# Autodesk Inventor assembly: Frame
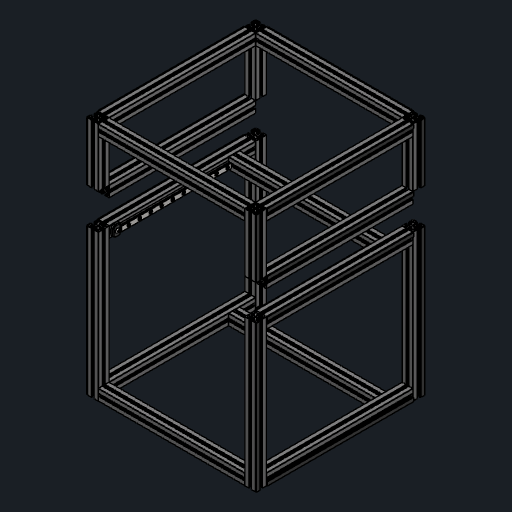
[picture p0: Inventor's stored thumbnail of the model, 512x512]
Saved by Autodesk Inventor 2026 (Build 300175050, 175E)
## iProperties
Created: 2025-05-09
Part Number: Frame
Document SubType Name: Assembly
Designer: AdminForWorker
Title: Frame
Author: AdminForWorker
## Documents named in this file (7)
- C:\Users\Joshua Eah\Documents\GitHub\Voron-0\CAD\Master Assembly\Frame\Frame.iam
- C:\Users\Joshua Eah\Documents\GitHub\Voron-0\CAD\Master Assembly\Linear Rail\MGN7 Rail 150mm.iam
- MGN7 150mm Rail.iam
- C:\Users\Joshua Eah\Documents\GitHub\Voron-0\CAD\Master Assembly\Frame\Subassemblies\Rail Stop.iam
- C:\Users\Joshua Eah\Documents\GitHub\Voron-0\CAD\Master Assembly\Frame\Subassemblies\Frame Extrusions.iam
- Extrusions.iam
- C:\Users\Joshua Eah\Documents\GitHub\Voron-0\CAD\Master Assembly\Frame\Foam Tape.iam
## Components (6 placed, 4 different names)
1. Extrusions:1 [sub-assembly]
2. MGN7 150mm Rail:3 [sub-assembly] — Mate:20
3. MGN7 150mm Rail:4 [sub-assembly] — Mate:22
4. Rail Stop:1 [sub-assembly] — Mate:20
5. Rail Stop:2 [sub-assembly] — Mate:22
6. Foam Tape:1 [sub-assembly]
## Relationships (99: Flush 62, Mate 37)
- [Mate]: Extrusions:1 ↔ MGN7 150mm Rail:3
- [Mate] (0.1 mm): Extrusions:1 ↔ MGN7 150mm Rail:3
- [Flush] (38 mm): Extrusions:1 ↔ MGN7 150mm Rail:3
- [Flush] (38 mm): Extrusions:1 ↔ MGN7 150mm Rail:4
- [Mate]: Extrusions:1 ↔ MGN7 150mm Rail:4
- [Mate] (0.1 mm): Extrusions:1 ↔ MGN7 150mm Rail:4
- [Mate]: Extrusions:1 ↔ Rail Stop:1
- Mate:20: MGN7 150mm Rail:3 ↔ Rail Stop:1
- [Flush]: Extrusions:1 ↔ Rail Stop:1
- [Mate]: Extrusions:1 ↔ Rail Stop:2
- Mate:22: MGN7 150mm Rail:4 ↔ Rail Stop:2
- [Flush]: Extrusions:1 ↔ Rail Stop:2
- [Mate]: Extrusions:1 ↔ Foam Tape:1
- [Flush]: Extrusions:1 ↔ Foam Tape:1
- [Mate]: Extrusions:1 ↔ Foam Tape:1
- [Flush]: Extrusions:1 ↔ Foam Tape:1
- [Mate]: Extrusions:1 ↔ Foam Tape:1
- [Flush]: Extrusions:1 ↔ Foam Tape:1
- [Mate]: Extrusions:1 ↔ Foam Tape:1
- [Flush]: Extrusions:1 ↔ Foam Tape:1
- [Mate]: Extrusions:1 ↔ Foam Tape:1
- [Flush]: Extrusions:1 ↔ Foam Tape:1
- [Flush]: Extrusions:1 ↔ Foam Tape:1
- [Mate]: Extrusions:1 ↔ Foam Tape:1
- [Flush]: Extrusions:1 ↔ Foam Tape:1
- [Flush]: Extrusions:1 ↔ Foam Tape:1
- [Mate]: Extrusions:1 ↔ Foam Tape:1
- [Flush]: Extrusions:1 ↔ Foam Tape:1
- [Flush]: Extrusions:1 ↔ Foam Tape:1
- [Mate]: Extrusions:1 ↔ Foam Tape:1
- [Flush]: Extrusions:1 ↔ Foam Tape:1
- [Flush]: Extrusions:1 ↔ Foam Tape:1
- [Mate]: Extrusions:1 ↔ Foam Tape:1
- [Flush]: Extrusions:1 ↔ Foam Tape:1
- [Flush]: Extrusions:1 ↔ Foam Tape:1
- [Mate]: Extrusions:1 ↔ Foam Tape:1
- [Flush]: Extrusions:1 ↔ Foam Tape:1
- [Flush]: Extrusions:1 ↔ Foam Tape:1
- [Mate]: Extrusions:1 ↔ Foam Tape:1
- [Flush]: Extrusions:1 ↔ Foam Tape:1
- [Flush]: Extrusions:1 ↔ Foam Tape:1
- [Mate]: Extrusions:1 ↔ Foam Tape:1
- [Flush]: Extrusions:1 ↔ Foam Tape:1
- [Flush]: Extrusions:1 ↔ Foam Tape:1
- [Flush]: Extrusions:1 ↔ Foam Tape:1
- [Flush]: Extrusions:1 ↔ Foam Tape:1
- [Mate]: Extrusions:1 ↔ Foam Tape:1
- [Flush]: Extrusions:1 ↔ Foam Tape:1
- [Flush]: Extrusions:1 ↔ Foam Tape:1
- [Mate]: Extrusions:1 ↔ Foam Tape:1
- [Flush]: Extrusions:1 ↔ Foam Tape:1
- [Flush]: Extrusions:1 ↔ Foam Tape:1
- [Flush]: Extrusions:1 ↔ Foam Tape:1
- [Flush]: Extrusions:1 ↔ Foam Tape:1
- [Mate]: Extrusions:1 ↔ Foam Tape:1
- [Flush]: Extrusions:1 ↔ Foam Tape:1
- [Flush]: Extrusions:1 ↔ Foam Tape:1
- [Mate]: Extrusions:1 ↔ Foam Tape:1
- [Flush]: Extrusions:1 ↔ Foam Tape:1
- [Flush]: Extrusions:1 ↔ Foam Tape:1
- [Mate]: Extrusions:1 ↔ Foam Tape:1
- [Flush]: Extrusions:1 ↔ Foam Tape:1
- [Flush]: Extrusions:1 ↔ Foam Tape:1
- [Mate]: Extrusions:1 ↔ Foam Tape:1
- [Flush]: Extrusions:1 ↔ Foam Tape:1
- [Flush]: Extrusions:1 ↔ Foam Tape:1
- [Mate]: Extrusions:1 ↔ Foam Tape:1
- [Flush]: Extrusions:1 ↔ Foam Tape:1
- [Flush]: Extrusions:1 ↔ Foam Tape:1
- [Mate]: Extrusions:1 ↔ Foam Tape:1
- [Flush]: Extrusions:1 ↔ Foam Tape:1
- [Flush]: Extrusions:1 ↔ Foam Tape:1
- [Mate]: Extrusions:1 ↔ Foam Tape:1
- [Flush]: Extrusions:1 ↔ Foam Tape:1
- [Flush]: Extrusions:1 ↔ Foam Tape:1
- [Mate]: Extrusions:1 ↔ Foam Tape:1
- [Flush]: Extrusions:1 ↔ Foam Tape:1
- [Flush]: Extrusions:1 ↔ Foam Tape:1
- [Mate]: Extrusions:1 ↔ Foam Tape:1
- [Flush]: Extrusions:1 ↔ Foam Tape:1
- [Flush]: Extrusions:1 ↔ Foam Tape:1
- [Mate]: Extrusions:1 ↔ Foam Tape:1
- [Flush]: Extrusions:1 ↔ Foam Tape:1
- [Flush]: Extrusions:1 ↔ Foam Tape:1
- [Mate]: Extrusions:1 ↔ Foam Tape:1
- [Flush]: Extrusions:1 ↔ Foam Tape:1
- [Flush]: Extrusions:1 ↔ Foam Tape:1
- [Mate]: Extrusions:1 ↔ Foam Tape:1
- [Flush]: Extrusions:1 ↔ Foam Tape:1
- [Flush]: Extrusions:1 ↔ Foam Tape:1
- [Mate]: Extrusions:1 ↔ Foam Tape:1
- [Flush]: Extrusions:1 ↔ Foam Tape:1
- [Flush]: Extrusions:1 ↔ Foam Tape:1
- [Mate]: Extrusions:1 ↔ Foam Tape:1
- [Flush]: Extrusions:1 ↔ Foam Tape:1
- [Flush]: Extrusions:1 ↔ Foam Tape:1
- [Mate]: Extrusions:1 ↔ Foam Tape:1
- [Flush]: Extrusions:1 ↔ Foam Tape:1
- [Flush]: Extrusions:1 ↔ Foam Tape:1
